# Autodesk Inventor assembly: FrontLink
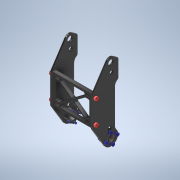
[picture p0: Inventor's stored thumbnail of the model, 180x180]
Saved by Autodesk Inventor 2022 (Build 260153000, 153)
## iProperties
Created: 2022-06-15
Part Number: FrontLink
Document SubType Name: Assembly
Designer: Masato Kubotera
Author: Masato Kubotera
## Documents named in this file (7)
- C:\Users\MasatoKubotera\Documents\Inventor\SUSTAINA-OP\LowerBody\Link\FrontLink.iam
- C:\Users\MasatoKubotera\Documents\Inventor\SUSTAINA-OP\LowerBody\Link\FrontLink_diagonal.ipt
- C:\Users\MasatoKubotera\Documents\Inventor\SUSTAINA-OP\LowerBody\Link\FrontLink_frame.ipt
- C:\Users\MasatoKubotera\Documents\Inventor\SUSTAINA-OP\ReadyMade\Washer\WSSS-12-10-8.ipt
- C:\Users\MasatoKubotera\Documents\Inventor\SUSTAINA-OP\LowerBody\Knee\Knee_clamp.ipt
- C:\Users\MasatoKubotera\Documents\Inventor\SUSTAINA-OP\ReadyMade\Screw\UC-2610.ipt
- C:\Users\MasatoKubotera\Documents\Inventor\SUSTAINA-OP\ReadyMade\Screw\UC-0306.ipt
## Components (19 placed, 6 different names)
1. FrontLink_diagonal:1 — 挿入:1, 挿入:3, 挿入:4, 挿入:6
2. FrontLink_frame:1 — 挿入:1, 挿入:3, 挿入:9, 挿入:10, 挿入:11, 挿入:12, 挿入:17, 挿入:18, 挿入:19, 挿入:20, 挿入:25, 挿入:27, 対称度:1, メイト:2
3. FrontLink_frame:2 — 挿入:4, 挿入:6, 挿入:13, 挿入:14, 挿入:15, 挿入:16, 挿入:21, 挿入:22, 挿入:23, 挿入:24, 挿入:28, 挿入:30, 対称度:1
4. Knee_clamp:1 — 挿入:7, 挿入:9, 挿入:10, 挿入:11, 挿入:12
5. Knee_clamp:2 — 挿入:8, 挿入:13, 挿入:14, 挿入:15, 挿入:16
6. WSSS-12-10-8:1 — 挿入:7, メイト:3
7. WSSS-12-10-8:2 — 挿入:8
8. UC-2610:1 — 挿入:17
9. UC-2610:2 — 挿入:18
10. UC-2610:3 — 挿入:19
11. UC-2610:4 — 挿入:20
12. UC-2610:5 — 挿入:21
13. UC-2610:6 — 挿入:22
14. UC-2610:7 — 挿入:23
15. UC-2610:8 — 挿入:24
16. UC-0306:1 — 挿入:25
17. UC-0306:3 — 挿入:27
18. UC-0306:4 — 挿入:28
19. UC-0306:6 — 挿入:30
## Relationships (34: Insert 26, Mate 7, Symmetry 1)
- 挿入:1 [Insert]: FrontLink_diagonal:1 ↔ FrontLink_frame:1
- 挿入:3 [Insert]: FrontLink_diagonal:1 ↔ FrontLink_frame:1
- 挿入:4 [Insert]: FrontLink_diagonal:1 ↔ FrontLink_frame:2
- 挿入:6 [Insert]: FrontLink_diagonal:1 ↔ FrontLink_frame:2
- 挿入:7 [Insert]: Knee_clamp:1 ↔ WSSS-12-10-8:1
- 挿入:8 [Insert]: Knee_clamp:2 ↔ WSSS-12-10-8:2
- 挿入:9 [Insert]: FrontLink_frame:1 ↔ Knee_clamp:1
- 挿入:10 [Insert]: FrontLink_frame:1 ↔ Knee_clamp:1
- 挿入:11 [Insert]: FrontLink_frame:1 ↔ Knee_clamp:1
- 挿入:12 [Insert]: FrontLink_frame:1 ↔ Knee_clamp:1
- 挿入:13 [Insert]: FrontLink_frame:2 ↔ Knee_clamp:2
- 挿入:14 [Insert]: FrontLink_frame:2 ↔ Knee_clamp:2
- 挿入:15 [Insert]: FrontLink_frame:2 ↔ Knee_clamp:2
- 挿入:16 [Insert]: FrontLink_frame:2 ↔ Knee_clamp:2
- 挿入:17 [Insert]: FrontLink_frame:1 ↔ UC-2610:1
- 挿入:18 [Insert]: FrontLink_frame:1 ↔ UC-2610:2
- 挿入:19 [Insert]: FrontLink_frame:1 ↔ UC-2610:3
- 挿入:20 [Insert]: FrontLink_frame:1 ↔ UC-2610:4
- 挿入:21 [Insert]: FrontLink_frame:2 ↔ UC-2610:5
- 挿入:22 [Insert]: FrontLink_frame:2 ↔ UC-2610:6
- 挿入:23 [Insert]: FrontLink_frame:2 ↔ UC-2610:7
- 挿入:24 [Insert]: FrontLink_frame:2 ↔ UC-2610:8
- 挿入:25 [Insert]: FrontLink_frame:1 ↔ UC-0306:1
- 挿入:27 [Insert]: FrontLink_frame:1 ↔ UC-0306:3
- 挿入:28 [Insert]: FrontLink_frame:2 ↔ UC-0306:4
- 挿入:30 [Insert]: FrontLink_frame:2 ↔ UC-0306:6
- 対称度:1 [Symmetry]: FrontLink_frame:1 ↔ FrontLink_frame:2
- メイト:1 [Mate]
- メイト:2 [Mate]: FrontLink_frame:1
- メイト:3 [Mate]: WSSS-12-10-8:1
- メイト:4 [Mate]
- メイト:5 [Mate]
- メイト:6 [Mate]
- メイト:7 [Mate]
